# Autodesk Inventor assembly: sonda_obudowa
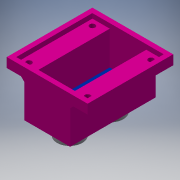
[picture p0: Inventor's stored thumbnail of the model, 180x180]
Saved by Autodesk Inventor 2019 (Build 230136000, 136)
## iProperties
Created: 2019-08-12
Part Number: sonda_obudowa
Material: Ogólny
Document SubType Name: Assembly
Designer: mikol
Author: mikol
## Documents named in this file (3)
- C:\Users\mikol\Desktop\Projekty\Pomiar_poziomu_wody\pomiar\projekt_obudowy\sonda_obudowa.iam
- C:\Users\mikol\Desktop\Projekty\Pomiar_poziomu_wody\pomiar\projekt_obudowy\obudowa_baza.ipt
- C:\Users\mikol\Desktop\Projekty\Pomiar_poziomu_wody\pomiar\projekt_obudowy\ultrasonicUser Library-PING ultrasonic distance sensor.ipt
## Components (2 placed, 2 different names)
1. obudowa_baza:1 — Rigid:1
2. ultrasonicUser Library-PING ultrasonic distance sensor:1 — Rigid:1
## Relationships (1: WeldJoint 1)
- Rigid:1 [WeldJoint] (6 mm): obudowa_baza:1 ↔ ultrasonicUser Library-PING ultrasonic distance sensor:1
